# Autodesk Inventor assembly: X-Gantry Joiner Left V4 Assembly
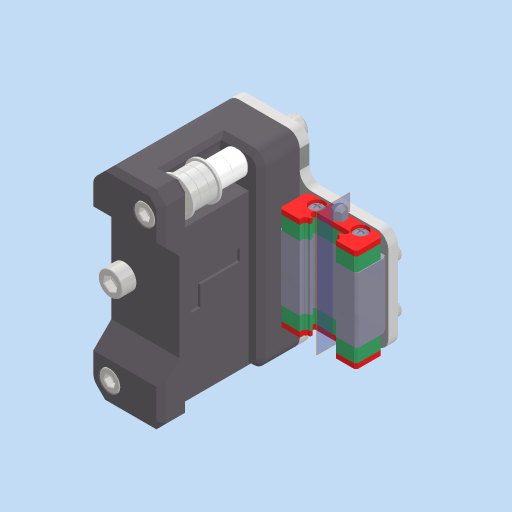
[picture p0: Inventor's stored thumbnail of the model, 512x512]
Saved by Autodesk Inventor 2023.2 (Build 272271000, 271)
## iProperties
Created: 2024-02-08
Part Number: X-Gantry Joiner Left V4 Assembly
Document SubType Name: Assembly
Designer: Nils Bade
Author: Nils Bade
## Documents named in this file (18)
- C:\Users\nilsb\Documents\Inventor\Projektarbeit-Bade\RatRig_Bade\X-Gantry Joiner Left V4 Assembly.iam
- C:\Users\nilsb\Documents\Inventor\Projektarbeit-Bade\RatRig_modified\xy Joiner Left for 4040 V3.ipt
- C:\Users\nilsb\Documents\Inventor\Projektarbeit-Bade\RatRig_modified\XY Joiner Plate for 4040 V3.ipt
- C:\Users\nilsb\Documents\Inventor\Projektarbeit-Bade\RatRig_modified\MGN15 Linear-Rail-Block.ipt
- C:\Users\nilsb\Documents\Inventor\Projektarbeit-Bade\Schrauben\Cap Head Screw M5x60.ipt
- C:\Users\nilsb\Documents\Inventor\Projektarbeit-Bade\RatRig_Standards\Hex Locking Nut - M5 v2.ipt
- C:\Users\nilsb\Documents\Inventor\Projektarbeit-Bade\Schrauben\Cap Head Screw M6x16.ipt
- C:\Users\nilsb\Documents\Inventor\Projektarbeit-Bade\Schrauben\Cap Head Screw M6x12 v2.ipt
- C:\Users\nilsb\Documents\Inventor\Projektarbeit-Bade\RatRig_modified\T-NUT - DropIn 4040 SERIES - M6.ipt
- C:\Users\nilsb\Documents\Inventor\Projektarbeit-Bade\RatRig_Standards\Mini Precision Shim - 8x5x1mm v2.ipt
- C:\Users\nilsb\Documents\Inventor\Projektarbeit-Bade\RatRig_Standards\Ball Bearing - F695ZZ v1.ipt
- C:\Users\nilsb\Documents\Inventor\Projektarbeit-Bade\RatRig_Standards\Ball Bearing - 695ZZ v1.ipt
- C:\Users\nilsb\Documents\Inventor\Projektarbeit-Bade\RatRig_Standards\Aluminium Spacer - 6mm v2.ipt
- C:\Users\nilsb\Documents\Inventor\Projektarbeit-Bade\Schrauben\Cap Head Screw M3x8 v2.ipt
- C:\Users\nilsb\Documents\Inventor\Projektarbeit-Bade\RatRig_modified\X-Gantry Enstop Mount.ipt
- C:\Users\nilsb\Documents\Inventor\Projektarbeit-Bade\Schrauben\Cap Head Screw M4x8 - DIN912.ipt
- C:\Users\nilsb\Documents\Inventor\Projektarbeit-Bade\RatRig_modified\Endstop-Horizontal-RatRig.ipt
- C:\Users\nilsb\Documents\Inventor\Projektarbeit-Bade\RatRig_Standards\Hex Locking Nut - M3 v2.ipt
## Components (39 placed, 17 different names)
1. xy Joiner Left for 4040 V3:1 — Passend:1, Passend:2, Passend:3, Passend:4, Passend:27, Passend:28, Winkel:1, Winkel:2, Passend:31, Passend:32, Passend:50, Passend:51, Passend:52, Passend:70, Passend:71, Passend:72, Passend:73
2. XY Joiner Plate for 4040 V3:1 — Passend:1, Passend:2, Passend:3, Passend:4, Passend:5, Passend:6, Passend:7, Passend:8, Passend:25, Passend:26, Passend:49, Passend:69, Passend:75, Passend:76, Passend:77, Winkel:3, Winkel:4, Winkel:5, Fluchtend:1
3. MGN15 Linear-Rail-Block:1 — Passend:5, Passend:6, Passend:7, Passend:8
4. Cap Head Screw M3x8 v2:1
5. Cap Head Screw M3x8 v2:2
6. Cap Head Screw M3x8 v2:3
7. Cap Head Screw M3x8 v2:4
8. Cap Head Screw M6x16:1 — Passend:25, Passend:26, Passend:29
9. Cap Head Screw M6x12 v2:1 — Passend:27, Passend:28, Passend:30
10. T-NUT - DROP IN TYPE FOR 40 SERIES - M6:1 — Passend:29, Winkel:2, Passend:31
11. T-NUT - DROP IN TYPE FOR 40 SERIES - M6:2 — Passend:30, Winkel:1, Passend:32
12. Cap Head Screw M5x60:1 — Passend:50, Passend:52
13. Hex Locking Nut - M5 v2:1 — Passend:49
14. Mini Precision Shim - 8x5x1mm v2:1
15. Mini Precision Shim - 8x5x1mm v2:2
16. Mini Precision Shim - 8x5x1mm v2:3 — Passend:51
17. Ball Bearing - F695ZZ v1:1
18. Ball Bearing - F695ZZ v1:2
19. Ball Bearing - 695ZZ v1:1
20. Aluminium Spacer - 6mm v2:1
21. Aluminium Spacer - 6mm v2:2
22. Cap Head Screw M5x60:2 — Passend:71, Passend:72
23. Hex Locking Nut - M5 v2:2 — Passend:69
24. Mini Precision Shim - 8x5x1mm v2:4
25. Mini Precision Shim - 8x5x1mm v2:5
26. Mini Precision Shim - 8x5x1mm v2:6 — Passend:70
27. Ball Bearing - F695ZZ v1:3
28. Ball Bearing - F695ZZ v1:4
29. Ball Bearing - 695ZZ v1:2
30. Aluminium Spacer - 6mm v2:3
31. Aluminium Spacer - 6mm v2:4
32. X-Gantry Enstop Mount:1 — Passend:73, Passend:75, Passend:78, Passend:79, Passend:80, Passend:81, Passend:82, Passend:83, Passend:86, Winkel:5, Fluchtend:1
33. Cap Head Screw M4x8 - DIN912:1 — Passend:76, Passend:78
34. Cap Head Screw M4x8 - DIN912:2 — Passend:77, Passend:79
35. Cap Head Screw M3x8 v2:5 — Passend:80, Passend:82, Passend:85, Passend:88
36. Cap Head Screw M3x8 v2:6 — Passend:81, Passend:83, Passend:84, Passend:87
37. Endstop-Horizontal-RatRig:1 — Passend:84, Passend:85, Passend:86, Passend:89, Passend:90
38. Hex Locking Nut - M3 v2:1 — Passend:87, Passend:90, Winkel:3
39. Hex Locking Nut - M3 v2:2 — Passend:88, Passend:89, Winkel:4
## Relationships (87: Mate 81, Angle 5, Flush 1)
- Passend:1 [Mate]: xy Joiner Left for 4040 V3:1 ↔ XY Joiner Plate for 4040 V3:1
- Passend:2 [Mate]: xy Joiner Left for 4040 V3:1 ↔ XY Joiner Plate for 4040 V3:1
- Passend:3 [Mate]: xy Joiner Left for 4040 V3:1 ↔ XY Joiner Plate for 4040 V3:1
- Passend:4 [Mate]: xy Joiner Left for 4040 V3:1 ↔ XY Joiner Plate for 4040 V3:1
- Passend:5 [Mate]: XY Joiner Plate for 4040 V3:1 ↔ MGN15 Linear-Rail-Block:1
- Passend:6 [Mate]: XY Joiner Plate for 4040 V3:1 ↔ MGN15 Linear-Rail-Block:1
- Passend:7 [Mate]: XY Joiner Plate for 4040 V3:1 ↔ MGN15 Linear-Rail-Block:1
- Passend:8 [Mate]: XY Joiner Plate for 4040 V3:1 ↔ MGN15 Linear-Rail-Block:1
- [Mate]: XY Joiner Plate for 4040 V3:1 ↔ Cap Head Screw M3x8 v2:4
- [Mate]: XY Joiner Plate for 4040 V3:1 ↔ Cap Head Screw M3x8 v2:1
- [Mate]: XY Joiner Plate for 4040 V3:1 ↔ Cap Head Screw M3x8 v2:2
- [Mate]: XY Joiner Plate for 4040 V3:1 ↔ Cap Head Screw M3x8 v2:3
- [Mate]: XY Joiner Plate for 4040 V3:1 ↔ Cap Head Screw M3x8 v2:4
- [Mate]: XY Joiner Plate for 4040 V3:1 ↔ Cap Head Screw M3x8 v2:1
- [Mate]: XY Joiner Plate for 4040 V3:1 ↔ Cap Head Screw M3x8 v2:2
- [Mate]: XY Joiner Plate for 4040 V3:1 ↔ Cap Head Screw M3x8 v2:3
- Passend:25 [Mate]: XY Joiner Plate for 4040 V3:1 ↔ Cap Head Screw M6x16:1
- Passend:26 [Mate]: XY Joiner Plate for 4040 V3:1 ↔ Cap Head Screw M6x16:1
- Passend:27 [Mate]: xy Joiner Left for 4040 V3:1 ↔ Cap Head Screw M6x12 v2:1
- Passend:28 [Mate]: xy Joiner Left for 4040 V3:1 ↔ Cap Head Screw M6x12 v2:1
- Passend:29 [Mate]: Cap Head Screw M6x16:1 ↔ T-NUT - DROP IN TYPE FOR 40 SERIES - M6:1
- Passend:30 [Mate]: Cap Head Screw M6x12 v2:1 ↔ T-NUT - DROP IN TYPE FOR 40 SERIES - M6:2
- Winkel:1 [Angle] (0 deg): xy Joiner Left for 4040 V3:1 ↔ T-NUT - DROP IN TYPE FOR 40 SERIES - M6:2
- Winkel:2 [Angle] (0 deg): xy Joiner Left for 4040 V3:1 ↔ T-NUT - DROP IN TYPE FOR 40 SERIES - M6:1
- Passend:31 [Mate] (4.6 mm): xy Joiner Left for 4040 V3:1 ↔ T-NUT - DROP IN TYPE FOR 40 SERIES - M6:1
- Passend:32 [Mate] (4.6 mm): xy Joiner Left for 4040 V3:1 ↔ T-NUT - DROP IN TYPE FOR 40 SERIES - M6:2
- [Mate]: Cap Head Screw M5x60:1 ↔ Hex Locking Nut - M5 v2:1
- [Mate]: Cap Head Screw M5x60:1 ↔ Mini Precision Shim - 8x5x1mm v2:3
- [Mate]: Cap Head Screw M5x60:1 ↔ Ball Bearing - F695ZZ v1:2
- [Mate]: Mini Precision Shim - 8x5x1mm v2:3 ↔ Ball Bearing - F695ZZ v1:2
- [Mate]: Cap Head Screw M5x60:1 ↔ Ball Bearing - 695ZZ v1:1
- [Mate]: Ball Bearing - F695ZZ v1:2 ↔ Ball Bearing - 695ZZ v1:1
- [Mate]: Cap Head Screw M5x60:1 ↔ Ball Bearing - F695ZZ v1:1
- [Mate]: Ball Bearing - F695ZZ v1:1 ↔ Ball Bearing - 695ZZ v1:1
- [Mate]: Cap Head Screw M5x60:1 ↔ Mini Precision Shim - 8x5x1mm v2:2
- [Mate]: Mini Precision Shim - 8x5x1mm v2:2 ↔ Ball Bearing - F695ZZ v1:1
- [Mate]: Cap Head Screw M5x60:1 ↔ Aluminium Spacer - 6mm v2:1
- [Mate]: Mini Precision Shim - 8x5x1mm v2:2 ↔ Aluminium Spacer - 6mm v2:1
- [Mate]: Cap Head Screw M5x60:1 ↔ Aluminium Spacer - 6mm v2:2
- [Mate]: Aluminium Spacer - 6mm v2:1 ↔ Aluminium Spacer - 6mm v2:2
- [Mate]: Cap Head Screw M5x60:1 ↔ Mini Precision Shim - 8x5x1mm v2:1
- [Mate]: Mini Precision Shim - 8x5x1mm v2:1 ↔ Aluminium Spacer - 6mm v2:2
- Passend:49 [Mate]: XY Joiner Plate for 4040 V3:1 ↔ Hex Locking Nut - M5 v2:1
- Passend:50 [Mate]: xy Joiner Left for 4040 V3:1 ↔ Cap Head Screw M5x60:1
- Passend:51 [Mate]: xy Joiner Left for 4040 V3:1 ↔ Mini Precision Shim - 8x5x1mm v2:3
- Passend:52 [Mate]: xy Joiner Left for 4040 V3:1 ↔ Cap Head Screw M5x60:1
- [Mate]: Cap Head Screw M5x60:2 ↔ Hex Locking Nut - M5 v2:2
- [Mate]: Cap Head Screw M5x60:2 ↔ Mini Precision Shim - 8x5x1mm v2:4
- [Mate]: Cap Head Screw M5x60:2 ↔ Ball Bearing - F695ZZ v1:3
- [Mate]: Mini Precision Shim - 8x5x1mm v2:4 ↔ Ball Bearing - F695ZZ v1:3
- [Mate]: Cap Head Screw M5x60:2 ↔ Ball Bearing - 695ZZ v1:2
- [Mate]: Ball Bearing - F695ZZ v1:3 ↔ Ball Bearing - 695ZZ v1:2
- [Mate]: Cap Head Screw M5x60:2 ↔ Ball Bearing - F695ZZ v1:4
- [Mate]: Ball Bearing - F695ZZ v1:4 ↔ Ball Bearing - 695ZZ v1:2
- [Mate]: Cap Head Screw M5x60:2 ↔ Mini Precision Shim - 8x5x1mm v2:5
- [Mate]: Mini Precision Shim - 8x5x1mm v2:5 ↔ Ball Bearing - F695ZZ v1:4
- [Mate]: Cap Head Screw M5x60:2 ↔ Aluminium Spacer - 6mm v2:3
- [Mate]: Mini Precision Shim - 8x5x1mm v2:5 ↔ Aluminium Spacer - 6mm v2:3
- [Mate]: Cap Head Screw M5x60:2 ↔ Aluminium Spacer - 6mm v2:4
- [Mate]: Aluminium Spacer - 6mm v2:3 ↔ Aluminium Spacer - 6mm v2:4
- [Mate]: Cap Head Screw M5x60:2 ↔ Mini Precision Shim - 8x5x1mm v2:6
- [Mate]: Mini Precision Shim - 8x5x1mm v2:6 ↔ Aluminium Spacer - 6mm v2:4
- Passend:69 [Mate]: XY Joiner Plate for 4040 V3:1 ↔ Hex Locking Nut - M5 v2:2
- Passend:70 [Mate]: xy Joiner Left for 4040 V3:1 ↔ Mini Precision Shim - 8x5x1mm v2:6
- Passend:71 [Mate]: xy Joiner Left for 4040 V3:1 ↔ Cap Head Screw M5x60:2
- Passend:72 [Mate]: xy Joiner Left for 4040 V3:1 ↔ Cap Head Screw M5x60:2
- Passend:73 [Mate]: xy Joiner Left for 4040 V3:1 ↔ X-Gantry Enstop Mount:1
- Passend:75 [Mate]: XY Joiner Plate for 4040 V3:1 ↔ X-Gantry Enstop Mount:1
- Passend:76 [Mate]: XY Joiner Plate for 4040 V3:1 ↔ Cap Head Screw M4x8 - DIN912:1
- Passend:77 [Mate]: XY Joiner Plate for 4040 V3:1 ↔ Cap Head Screw M4x8 - DIN912:2
- Passend:78 [Mate]: X-Gantry Enstop Mount:1 ↔ Cap Head Screw M4x8 - DIN912:1
- Passend:79 [Mate]: X-Gantry Enstop Mount:1 ↔ Cap Head Screw M4x8 - DIN912:2
- Passend:80 [Mate]: X-Gantry Enstop Mount:1 ↔ Cap Head Screw M3x8 v2:5
- Passend:81 [Mate]: X-Gantry Enstop Mount:1 ↔ Cap Head Screw M3x8 v2:6
- Passend:82 [Mate]: X-Gantry Enstop Mount:1 ↔ Cap Head Screw M3x8 v2:5
- Passend:83 [Mate]: X-Gantry Enstop Mount:1 ↔ Cap Head Screw M3x8 v2:6
- Passend:84 [Mate]: Cap Head Screw M3x8 v2:6 ↔ Endstop-Horizontal-RatRig:1
- Passend:85 [Mate]: Cap Head Screw M3x8 v2:5 ↔ Endstop-Horizontal-RatRig:1
- Passend:86 [Mate]: X-Gantry Enstop Mount:1 ↔ Endstop-Horizontal-RatRig:1
- Passend:87 [Mate]: Cap Head Screw M3x8 v2:6 ↔ Hex Locking Nut - M3 v2:1
- Passend:88 [Mate]: Cap Head Screw M3x8 v2:5 ↔ Hex Locking Nut - M3 v2:2
- Passend:89 [Mate]: Endstop-Horizontal-RatRig:1 ↔ Hex Locking Nut - M3 v2:2
- Passend:90 [Mate]: Endstop-Horizontal-RatRig:1 ↔ Hex Locking Nut - M3 v2:1
- Winkel:3 [Angle] (0 deg): XY Joiner Plate for 4040 V3:1 ↔ Hex Locking Nut - M3 v2:1
- Winkel:4 [Angle] (0 deg): XY Joiner Plate for 4040 V3:1 ↔ Hex Locking Nut - M3 v2:2
- Winkel:5 [Angle] (0 deg): XY Joiner Plate for 4040 V3:1 ↔ X-Gantry Enstop Mount:1
- Fluchtend:1 [Flush] (-3 mm): XY Joiner Plate for 4040 V3:1 ↔ X-Gantry Enstop Mount:1
## Named parameters: d5_d37 = 0 mm, d8_d40 = 0 mm, d9_d42 = 0 mm, d10_d43 = 0 mm, d11_d44 = 0 mm, d79_d66 = 0 mm, d80_d67 = 0 mm, d81_d68 = 0 mm, d82_d69 = 0 mm
